# Autodesk Inventor assembly: Robot B
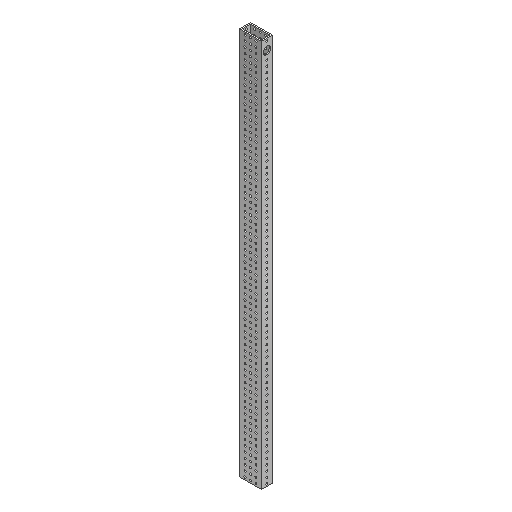
[picture p0: Inventor's stored thumbnail of the model, 512x512]
Saved by Autodesk Inventor 2025.3 (Build 293356000, 356)
## iProperties
Created: 2026-05-13
Part Number: Robot B
Document SubType Name: Assembly
Designer: djair.oliveira
Author: djair.oliveira
## Documents named in this file (2)
- C:\Users\djair.oliveira\Documents\GitHub\MT_2026\CAD\Model B\Robot B.iam
- C:\Users\djair.oliveira\Documents\GitHub\MT_2026\CAD\Model B\Elevador\Elevador.iam
## Components (1 placed, 1 different names)
1. Elevador:1 [sub-assembly] — Coincidente:6
## Relationships (1: Mate 1)
- Coincidente:6 [Mate] (76.2 mm): Elevador:1
